# Autodesk Inventor assembly: AM Shifter
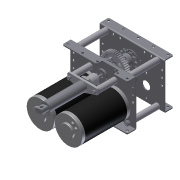
[picture p0: Inventor's stored thumbnail of the model, 180x180]
Saved by Autodesk Inventor 2011 (Build 150239000, 239)
## iProperties
Created: 2012-06-03
Part Number: AM Shifter
Document SubType Name: Assembly
Designer: Nemo
Author: Nemo
## Documents named in this file (11)
- H:\Nemo\Documents\Robotics\COTS Parts\Gearboxes\AM Shifter.iam
- H:\Nemo\Documents\Robotics\COTS Parts\Gearboxes\Housings\AM Shifter Inside Motor Plate.ipt
- H:\Nemo\Documents\Robotics\COTS Parts\Gearboxes\Housings\AM Shifter Outside Plate.ipt
- H:\Nemo\Documents\Robotics\COTS Parts\Gearboxes\Shafts\AM Shifter Cluster Shaft subassembly.iam
- H:\Nemo\Documents\Robotics\COTS Parts\Gearboxes\Shafts\AM Shifter Output Shaft subassembly.iam
- H:\Nemo\Documents\Robotics\COTS Parts\Motors\CIM motor 12T for AM Shifters.iam
- H:\Nemo\Documents\Robotics\COTS Parts\Gearboxes\Housings\AM Shifter Spacer.ipt
- H:\Nemo\Documents\Robotics\COTS Parts\Fasteners\10-32 SHCS x3000.ipt
- H:\Nemo\Documents\Robotics\COTS Parts\Fasteners\10-32 locknut.ipt
- H:\Nemo\Documents\Robotics\COTS Parts\Gearboxes\Shifters\Shifter Cylinder Subassembly.iam
- H:\Nemo\Documents\Robotics\COTS Parts\Fasteners\10-32 SHCS x625.ipt
## Components (25 placed, 10 different names)
1. AM Shifter Inside Motor Plate:1 — Mate:1, Mate:2, Mate:3, Insert:1, Insert:2, Insert:4, Insert:5, Mate:5, Mate:6, Insert:14, Insert:15, Insert:16, Insert:17, Insert:18, Mate:7, Insert:19, Insert:20, Insert:21, Insert:22, Insert:23, Insert:24
2. AM Shifter Outside Plate:1 — Mate:1, Mate:2, Mate:3, Insert:6, Insert:7, Insert:8, Insert:9, Insert:10, Insert:11, Insert:12, Insert:13
3. AM Shifter Cluster Shaft subassembly:1 [sub-assembly] — Insert:1
4. AM Shifter Output Shaft subassembly:1 [sub-assembly] — Insert:2
5. CIM motor 12T for AM Shifters:1 [sub-assembly] — Insert:4, Mate:6
6. CIM motor 12T for AM Shifters:2 [sub-assembly] — Insert:5, Mate:5
7. AM Shifter Spacer:1 — Insert:9
8. AM Shifter Spacer:2 — Insert:8
9. AM Shifter Spacer:3 — Insert:7
10. AM Shifter Spacer:4 — Insert:6
11. 10-32 SHCS x3000:1 — Insert:13
12. 10-32 SHCS x3000:2 — Insert:12
13. 10-32 SHCS x3000:3 — Insert:11
14. 10-32 SHCS x3000:4 — Insert:10
15. 10-32 locknut:1 — Insert:17
16. 10-32 locknut:2 — Insert:16
17. 10-32 locknut:3 — Insert:15
18. 10-32 locknut:4 — Insert:14
19. Shifter Cylinder Subassembly:1 [sub-assembly] — Insert:18, Mate:7
20. 10-32 locknut:5 — Insert:19
21. 10-32 locknut:6 — Insert:20
22. 10-32 SHCS x625:1 — Insert:21
23. 10-32 SHCS x625:2 — Insert:22
24. 10-32 SHCS x625:3 — Insert:24
25. 10-32 SHCS x625:4 — Insert:23
## Relationships (29: Insert 23, Mate 6)
- Mate:1: AM Shifter Inside Motor Plate:1 ↔ AM Shifter Outside Plate:1
- Mate:2: AM Shifter Inside Motor Plate:1 ↔ AM Shifter Outside Plate:1
- Mate:3 (66.04 mm): AM Shifter Inside Motor Plate:1 ↔ AM Shifter Outside Plate:1
- Insert:1: AM Shifter Inside Motor Plate:1 ↔ AM Shifter Cluster Shaft subassembly:1
- Insert:2: AM Shifter Inside Motor Plate:1 ↔ AM Shifter Output Shaft subassembly:1
- Insert:4: AM Shifter Inside Motor Plate:1 ↔ CIM motor 12T for AM Shifters:1
- Insert:5: AM Shifter Inside Motor Plate:1 ↔ CIM motor 12T for AM Shifters:2
- Mate:5: AM Shifter Inside Motor Plate:1 ↔ CIM motor 12T for AM Shifters:2
- Mate:6: AM Shifter Inside Motor Plate:1 ↔ CIM motor 12T for AM Shifters:1
- Insert:6: AM Shifter Outside Plate:1 ↔ AM Shifter Spacer:4
- Insert:7: AM Shifter Outside Plate:1 ↔ AM Shifter Spacer:3
- Insert:8: AM Shifter Outside Plate:1 ↔ AM Shifter Spacer:2
- Insert:9: AM Shifter Outside Plate:1 ↔ AM Shifter Spacer:1
- Insert:10: AM Shifter Outside Plate:1 ↔ 10-32 SHCS x3000:4
- Insert:11: AM Shifter Outside Plate:1 ↔ 10-32 SHCS x3000:3
- Insert:12: AM Shifter Outside Plate:1 ↔ 10-32 SHCS x3000:2
- Insert:13: AM Shifter Outside Plate:1 ↔ 10-32 SHCS x3000:1
- Insert:14: AM Shifter Inside Motor Plate:1 ↔ 10-32 locknut:4
- Insert:15: AM Shifter Inside Motor Plate:1 ↔ 10-32 locknut:3
- Insert:16: AM Shifter Inside Motor Plate:1 ↔ 10-32 locknut:2
- Insert:17: AM Shifter Inside Motor Plate:1 ↔ 10-32 locknut:1
- Insert:18: AM Shifter Inside Motor Plate:1 ↔ Shifter Cylinder Subassembly:1
- Mate:7: AM Shifter Inside Motor Plate:1 ↔ Shifter Cylinder Subassembly:1
- Insert:19: AM Shifter Inside Motor Plate:1 ↔ 10-32 locknut:5
- Insert:20: AM Shifter Inside Motor Plate:1 ↔ 10-32 locknut:6
- Insert:21: AM Shifter Inside Motor Plate:1 ↔ 10-32 SHCS x625:1
- Insert:22: AM Shifter Inside Motor Plate:1 ↔ 10-32 SHCS x625:2
- Insert:23: AM Shifter Inside Motor Plate:1 ↔ 10-32 SHCS x625:4
- Insert:24: AM Shifter Inside Motor Plate:1 ↔ 10-32 SHCS x625:3
